# Autodesk Inventor assembly: chassisassembly_foranalysis(cafa)
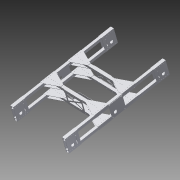
[picture p0: Inventor's stored thumbnail of the model, 180x180]
Saved by Autodesk Inventor 2015 SP1 (Build 190203100, 203)
## iProperties
Created: 2015-10-09
Part Number: chassisassembly_foranalysis(cafa)
Document SubType Name: Assembly
Designer: elilitwack
Mass: 5584.92 g
Surface Area: 19614.8 cm^2
Volume: 2068.49 cm^3
Density: 2.7 g/cm^3
Author: elilitwack
## Documents named in this file (12)
- C:\Users\elilitwack\Documents\2015 Offseason Chassis\West Coast Chassis Fall 2015\chassisassembly_foranalysis(cafa).iam
- C:\Users\elilitwack\Documents\2015 Offseason Chassis\West Coast Chassis Fall 2015\sideassembly(sa).iam
- C:\Users\elilitwack\Documents\2015 Offseason Chassis\West Coast Chassis Fall 2015\crossbar(cb).ipt
- C:\Users\elilitwack\Documents\2015 Offseason Chassis\West Coast Chassis Fall 2015\sideassembly(sa)_MIR.iam
- C:\Users\elilitwack\Documents\2015 Offseason Chassis\West Coast Chassis Fall 2015\cross_structural_plate(csp).ipt
- C:\Users\elilitwack\Documents\2015 Offseason Chassis\West Coast Chassis Fall 2015\bh_base.ipt
- C:\Users\elilitwack\Documents\2015 Offseason Chassis\West Coast Chassis Fall 2015\chassisassembly_foranalysis(cafa)\AIP\FEA\bl9pq4sm8.fins
- C:\Users\elilitwack\Documents\2015 Offseason Chassis\West Coast Chassis Fall 2015\chassisassembly_foranalysis(cafa)\AIP\FEA\bl9pq4sm8.fsat
- C:\Users\elilitwack\Documents\2015 Offseason Chassis\West Coast Chassis Fall 2015\chassisassembly_foranalysis(cafa)\AIP\FEA\bl9pq4sn4.ftes
- C:\Users\elilitwack\Documents\2015 Offseason Chassis\West Coast Chassis Fall 2015\chassisassembly_foranalysis(cafa)\AIP\FEA\bl9pq4sn4.fwiz
- C:\Users\elilitwack\Documents\2015 Offseason Chassis\West Coast Chassis Fall 2015\chassisassembly_foranalysis(cafa)\AIP\FEA\bl9pq4sxs.fmsh
- C:\Users\elilitwack\Documents\2015 Offseason Chassis\West Coast Chassis Fall 2015\chassisassembly_foranalysis(cafa)\AIP\FEA\bl9pq4sxt.fres
## Components (9 placed, 5 different names)
1. sideassembly(sa):1 [sub-assembly] — Mate:1, Mate:2, Mate:3, Mate:4, Mate:5, Mate:6, Mate:7, Mate:8, Mate:9, Mate:10, Mate:11, Mate:12
2. crossbar(cb):1 — Mate:1, Mate:2, Mate:3, Mate:21, Mate:22, Mate:24, Mate:31
3. crossbar(cb):2 — Mate:4, Mate:5, Mate:6, Mate:28, Mate:29, Mate:30
4. crossbar(cb):3 — Mate:10, Mate:11, Mate:12, Mate:13, Mate:14, Mate:15, Mate:23, Mate:25
5. crossbar(cb):4 — Mate:7, Mate:8, Mate:9, Mate:26, Mate:27
6. sideassembly(sa)_MIR:1 [sub-assembly] — Mate:13, Mate:14, Mate:15, Mate:23, Mate:24
7. cross_structural_plate(csp):1 — Mate:21, Mate:22, Mate:31
8. cross_structural_plate(csp):2 — Mate:25, Mate:26, Mate:27
9. bh_base:1 — Mate:28, Mate:29, Mate:30
## Relationships (26: Mate 26)
- Mate:1: sideassembly(sa):1 ↔ crossbar(cb):1
- Mate:2: sideassembly(sa):1 ↔ crossbar(cb):1
- Mate:3: sideassembly(sa):1 ↔ crossbar(cb):1
- Mate:4: sideassembly(sa):1 ↔ crossbar(cb):2
- Mate:5: sideassembly(sa):1 ↔ crossbar(cb):2
- Mate:6: sideassembly(sa):1 ↔ crossbar(cb):2
- Mate:7: sideassembly(sa):1 ↔ crossbar(cb):4
- Mate:8: sideassembly(sa):1 ↔ crossbar(cb):4
- Mate:9: sideassembly(sa):1 ↔ crossbar(cb):4
- Mate:10: sideassembly(sa):1 ↔ crossbar(cb):3
- Mate:11: sideassembly(sa):1 ↔ crossbar(cb):3
- Mate:12: sideassembly(sa):1 ↔ crossbar(cb):3
- Mate:13: crossbar(cb):3 ↔ sideassembly(sa)_MIR:1
- Mate:14: crossbar(cb):3 ↔ sideassembly(sa)_MIR:1
- Mate:15: crossbar(cb):3 ↔ sideassembly(sa)_MIR:1
- Mate:21: crossbar(cb):1 ↔ cross_structural_plate(csp):1
- Mate:22: crossbar(cb):1 ↔ cross_structural_plate(csp):1
- Mate:23: crossbar(cb):3 ↔ sideassembly(sa)_MIR:1
- Mate:24: crossbar(cb):1 ↔ sideassembly(sa)_MIR:1
- Mate:25: crossbar(cb):3 ↔ cross_structural_plate(csp):2
- Mate:26: crossbar(cb):4 ↔ cross_structural_plate(csp):2
- Mate:27: crossbar(cb):4 ↔ cross_structural_plate(csp):2
- Mate:28: crossbar(cb):2 ↔ bh_base:1
- Mate:29: crossbar(cb):2 ↔ bh_base:1
- Mate:30: crossbar(cb):2 ↔ bh_base:1
- Mate:31: crossbar(cb):1 ↔ cross_structural_plate(csp):1
## Named parameters: sa_3 = 271.524, sa_4 = -5177.66, sa_5 = -1269.22, sa_0 = 133447
note: some values were not read from the file. Shown as the stored number, unit unknown: "sa_3", "sa_4", "sa_5", "sa_0".
